# Autodesk Inventor assembly: 부피 구하기2
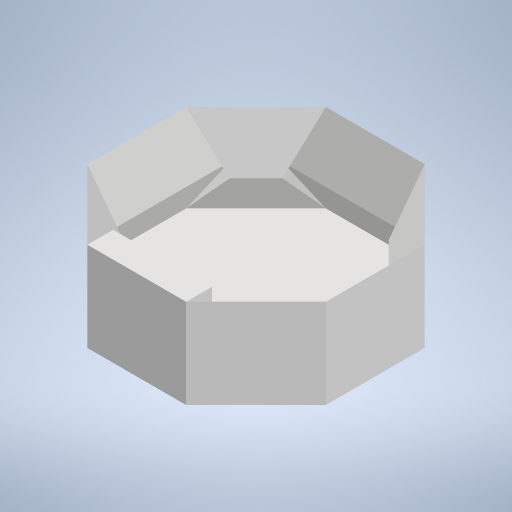
[picture p0: Inventor's stored thumbnail of the model, 512x512]
Saved by Autodesk Inventor 2024 (Build 280153000, 153)
## iProperties
Created: 2023-06-26
Part Number: 부피 구하기2
Document SubType Name: Assembly
Designer: jsw
Author: jsw
## Documents named in this file (3)
- C:\승원\co-op\OV-PAM\OV-PAM_modeling\부피 구하기2.iam
- C:\승원\co-op\OV-PAM\OV-PAM_modeling\부피 구하기2.ipt
- C:\승원\co-op\OV-PAM\OV-PAM_modeling\부피 구하기3.ipt
## Components (2 placed, 2 different names)
1. 부피 구하기2:1 — 플러쉬:1, 메이트:1, 메이트:2
2. 부피 구하기3:1 — 플러쉬:1, 메이트:1, 메이트:2
## Relationships (3: Mate 2, Flush 1)
- 플러쉬:1 [Flush]: 부피 구하기2:1 ↔ 부피 구하기3:1
- 메이트:1 [Mate]: 부피 구하기2:1 ↔ 부피 구하기3:1
- 메이트:2 [Mate]: 부피 구하기2:1 ↔ 부피 구하기3:1
